# Autodesk Inventor assembly: enix_assembly_v2
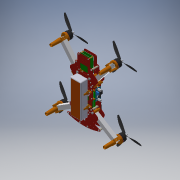
[picture p0: Inventor's stored thumbnail of the model, 180x180]
Saved by Autodesk Inventor 2016 (Build 200138000, 138)
## iProperties
Created: 2016-09-22
Part Number: enix_assembly_v2
Document SubType Name: Assembly
Designer: Jakub
Mass: 927.837 g
Surface Area: 3050.91 cm^2
Volume: 369.328 cm^3
Density: 2.51223 g/cm^3
Author: Jakub
## Documents named in this file (31)
- C:\Users\Jakub\Documents\DATA BANK\Projekty\Dron\Enix\V3\enix_assembly_v3.iam
- C:\Users\Jakub\Documents\DATA BANK\Projekty\Dron\Enix\V3\baseplate.ipt
- C:\Users\Jakub\Documents\DATA BANK\Projekty\Dron\Enix\V3\arm_grip.ipt
- C:\Users\Jakub\Documents\DATA BANK\Projekty\Dron\Enix\V3\arm_grip_mirror.ipt
- C:\Users\Jakub\Documents\DATA BANK\Projekty\Dron\Enix\V3\arm_lock.ipt
- C:\Users\Jakub\Documents\DATA BANK\Projekty\Dron\Enix\V3\dist25mm.ipt
- C:\Users\Jakub\Documents\Inventor\Content Center Files\R2016\en-US\AS 1427(04)\AS 1427 - M2 x 8(5) I.ipt
- C:\Users\Jakub\Documents\Inventor\Content Center Files\R2016\en-US\AS 1112 (2)\AS 1112 - M2  Type 5.ipt
- C:\Users\Jakub\Documents\DATA BANK\Projekty\Dron\Enix\V3\top_plate.ipt
- C:\Users\Jakub\Documents\Inventor\Content Center Files\R2016\en-US\UNI 6107\UNI 6107 - M4 x  30.ipt
- C:\Users\Jakub\Documents\Inventor\Content Center Files\R2016\en-US\ANSI B18.2.4.2M\ANSI B18.2.4.2M - M4x0,7 - 7.ipt
- C:\Users\Jakub\Documents\Inventor\Content Center Files\R2016\en-US\AS 1427(05)\AS 1427 - M3 x 5(5) II.ipt
- C:\Users\Jakub\Documents\DATA BANK\Projekty\Dron\Enix\V3\regulator.ipt
- C:\Users\Jakub\Documents\DATA BANK\Projekty\Dron\Enix\V3\dist10mmM2.ipt
- C:\Users\Jakub\Documents\DATA BANK\Projekty\Dron\Enix\V3\RASPBERRY PI 3.ipt
- C:\Users\Jakub\Documents\DATA BANK\Projekty\Dron\Enix\V3\dist5mmM2.ipt
- C:\Users\Jakub\Documents\DATA BANK\Projekty\Dron\Enix\V3\kamera.ipt
- C:\Users\Jakub\Documents\DATA BANK\Projekty\Dron\Enix\V3\cam_holder.ipt
- C:\Users\Jakub\Documents\DATA BANK\Projekty\Dron\Enix\V3\arm_front_rect.ipt
- C:\Users\Jakub\Documents\DATA BANK\Projekty\Dron\Enix\V3\arm_back_rect.ipt
- C:\Users\Jakub\Documents\DATA BANK\Projekty\Dron\Enix\V3\motor_mount.ipt
- C:\Users\Jakub\Documents\DATA BANK\Projekty\Dron\Enix\V3\motor_mount_lock.ipt
- C:\Users\Jakub\Documents\DATA BANK\Projekty\Dron\Enix\V3\Emax Rs2205 v1.ipt
- C:\Users\Jakub\Documents\DATA BANK\Projekty\Dron\Enix\V3\5x3_prop.ipt
- C:\Users\Jakub\Documents\DATA BANK\Projekty\Dron\Enix\V3\logic_conventer_lock.ipt
- C:\Users\Jakub\Documents\DATA BANK\Projekty\Dron\Enix\V3\altimuv3.iam
- C:\Users\Jakub\Documents\DATA BANK\Projekty\Dron\Enix\V3\kamamiLogicVoltageConverter\converter.iam
- C:\Users\Jakub\Documents\DATA BANK\Projekty\Dron\Enix\V3\kamamiTransformer\transformer.iam
- C:\Users\Jakub\Documents\DATA BANK\Projekty\Dron\Enix\V3\transformer_mount.ipt
- C:\Users\Jakub\Documents\DATA BANK\Projekty\Dron\Enix\V3\battery_distancer.ipt
- C:\Users\Jakub\Documents\DATA BANK\Projekty\Dron\Enix\V3\battery_vant_4500_4s.ipt
## Components (217 placed, 30 different names)
1. baseplate:1 — back_right_rot, front_right_rot, back_left_rot, front_left_rot, Mate:5, Mate:6, Mate:7, Mate:11, Mate:12, Mate:13, Mate:14, Mate:15, Mate:16, Mate:17, Mate:18, Mate:19, Mate:20, Mate:21, Mate:22, Mate:23, Mate:24, Mate:25, Mate:26, Mate:27, Mate:28, Mate:29, Mate:30, Mate:31, Mate:48, Mate:49, Mate:50, Mate:51, Mate:52, Mate:53, Mate:54, Mate:55, Mate:57, Mate:64, Mate:65, Mate:66, Mate:67, Mate:68, Mate:69, Mate:70, Mate:71, Mate:84, Mate:85, Mate:86, Mate:87, Mate:156, Mate:157, Mate:158, Mate:159, Mate:160, Mate:161, Mate:162, Mate:163, Mate:164, Mate:165, Mate:166, Mate:167, Mate:168, Mate:169, Mate:170, Mate:171, Mate:172, Mate:173, Mate:174, Mate:175, Mate:280, Mate:281, Mate:282, Mate:283, Mate:284, Mate:285, Mate:298, Mate:299, Mate:300, Mate:313, Mate:314, Mate:315, Mate:328, Mate:329, Mate:409, Mate:410, Mate:415, Mate:417, Mate:418, Mate:428, Mate:430, Mate:431, Mate:432, Mate:433, Mate:437, Mate:438, Mate:439, Mate:440, Mate:443, Mate:444, Mate:445, Mate:446, Mate:447, Mate:448, Mate:449, Mate:450, Mate:451, Mate:452, Mate:453, Mate:454, Mate:508, Mate:509, Mate:510, Mate:511, Mate:528, Mate:530, Mate:532, Mate:533, Mate:534, Mate:535, Mate:536, Mate:537, Mate:538, Mate:539, Mate:540, Mate:541, Mate:542, Mate:543, Mate:544, Mate:545
2. arm_grip:1 — back_right_rot, Mate:76, Mate:344, Mate:346, Angle:1
3. arm_grip:2 — front_right_rot, Mate:77, Mate:340, Mate:349, Angle:4
4. arm_grip_mirror:1 — back_left_rot, Mate:79, Mate:345, Mate:347, Angle:2
5. arm_grip_mirror:2 — front_left_rot, Mate:78, Mate:341, Mate:348, Angle:3
6. arm_lock:1 — Mate:5, Mate:6, Mate:7, Mate:32, Mate:33, Mate:38, Mate:39
7. arm_lock:2 — Mate:11, Mate:12, Mate:13, Mate:40, Mate:41, Mate:46, Mate:47
8. arm_lock:3 — Mate:14, Mate:15, Mate:16, Mate:42, Mate:43, Mate:44, Mate:45
9. arm_lock:4 — Mate:17, Mate:18, Mate:19, Mate:34, Mate:35, Mate:36, Mate:37
10. dist25mm:1 — Mate:20, Mate:23
11. dist25mm:2 — Mate:21, Mate:22
12. dist25mm:3 — Mate:27, Mate:28
13. dist25mm:4 — Mate:26, Mate:29
14. dist25mm:5 — Mate:25, Mate:30
15. dist25mm:6 — Mate:24, Mate:31, Mate:72, Mate:73
16. AS 1427 H - Metric M2 x 8:1 — Mate:32, Mate:38
17. AS 1427 H - Metric M2 x 8:2 — Mate:33, Mate:39, Mate:56
18. AS 1427 H - Metric M2 x 8:3 — Mate:34, Mate:36, Mate:63
19. AS 1427 H - Metric M2 x 8:4 — Mate:35, Mate:37, Mate:62
20. AS 1427 H - Metric M2 x 8:5 — Mate:42, Mate:44, Mate:60
21. AS 1427 H - Metric M2 x 8:6 — Mate:43, Mate:45, Mate:61
22. AS 1427 H - Metric M2 x 8:7 — Mate:41, Mate:46, Mate:58
23. AS 1427 H - Metric M2 x 8:8 — Mate:40, Mate:47, Mate:59
24. AS 1112 (2) - Metric M2  Type 5:1 — Mate:55, Mate:62
25. AS 1112 (2) - Metric M2  Type 5:2 — Mate:54, Mate:61
26. AS 1112 (2) - Metric M2  Type 5:3 — Mate:53, Mate:60
27. AS 1112 (2) - Metric M2  Type 5:4 — Mate:52, Mate:56
28. AS 1112 (2) - Metric M2  Type 5:5 — Mate:51, Mate:58
29. AS 1112 (2) - Metric M2  Type 5:6 — Mate:50, Mate:57
30. AS 1112 (2) - Metric M2  Type 5:7 — Mate:49, Mate:59
31. AS 1112 (2) - Metric M2  Type 5:8 — Mate:48, Mate:63
32. dist25mm:7 — Mate:68, Mate:69
33. dist25mm:8 — Mate:70, Mate:71, Mate:74
34. dist25mm:9 — Mate:66, Mate:67, Mate:75
35. dist25mm:10 — Mate:64, Mate:65
36. top_plate:1 — Mate:72, Mate:73, Mate:74, Mate:75, Mate:80, Mate:81, Mate:82, Mate:83, Mate:92, Mate:93, Mate:94, Mate:95, Mate:96, Mate:97, Mate:98, Mate:99, Mate:100, Mate:101, Mate:102, Mate:103, Mate:104, Mate:105, Mate:106, Mate:107, Mate:108, Mate:109, Mate:110, Mate:111, Mate:112, Mate:113, Mate:114, Mate:115, Mate:116, Mate:117, Mate:118, Mate:119, Mate:136, Mate:137, Mate:138, Mate:139, Mate:140, Mate:141, Mate:142, Mate:143, Mate:144, Mate:145, Mate:146, Mate:147, Mate:148, Mate:149, Mate:150, Mate:151, Mate:152, Mate:153, Mate:154, Mate:155, Mate:219, Mate:220, Mate:221, Mate:222, Mate:223, Mate:224, Mate:225, Mate:226, Mate:249, Mate:250, Mate:251, Mate:252, Mate:419, Mate:420, Mate:421, Mate:422, Mate:425, Mate:426, Mate:484, Mate:485, Mate:492, Mate:493, Mate:496, Mate:497, Mate:502, Mate:503, Mate:504, Mate:505
37. UNI 6107 M4 x  30:1 — Mate:76, Mate:81, Mate:89
38. UNI 6107 M4 x  30:2 — Mate:77, Mate:82, Mate:90
39. UNI 6107 M4 x  30:3 — Mate:78, Mate:83, Mate:91
40. UNI 6107 M4 x  30:4 — Mate:79, Mate:80, Mate:88
41. ANSI B18.2.4.2M M4x0,7:5 — Mate:87, Mate:91
42. ANSI B18.2.4.2M M4x0,7:6 — Mate:86, Mate:90
43. ANSI B18.2.4.2M M4x0,7:7 — Mate:85, Mate:88
44. ANSI B18.2.4.2M M4x0,7:8 — Mate:84, Mate:89
45. arm_lock:5 — Mate:92, Mate:93, Mate:94, Mate:132, Mate:133
46. arm_lock:6 — Mate:95, Mate:96, Mate:97, Mate:128, Mate:129
47. arm_lock:7 — Mate:98, Mate:99, Mate:100, Mate:120, Mate:121
48. arm_lock:8 — Mate:101, Mate:102, Mate:103, Mate:124, Mate:125
49. AS 1427 H - Metric M2 x 8:9 — Mate:108, Mate:118, Mate:131
50. AS 1427 H - Metric M2 x 8:10 — Mate:107, Mate:113, Mate:127
51. AS 1427 H - Metric M2 x 8:11 — Mate:109, Mate:119, Mate:130
52. AS 1427 H - Metric M2 x 8:12 — Mate:106, Mate:112, Mate:126
53. AS 1427 H - Metric M2 x 8:13 — Mate:110, Mate:117, Mate:135
54. AS 1427 H - Metric M2 x 8:14 — Mate:105, Mate:114, Mate:123
55. AS 1427 H - Metric M2 x 8:15 — Mate:111, Mate:116, Mate:134
56. AS 1427 H - Metric M2 x 8:16 — Mate:104, Mate:115, Mate:122
57. AS 1112 (2) - Metric M2  Type 5:9 — Mate:120, Mate:123
58. AS 1112 (2) - Metric M2  Type 5:10 — Mate:121, Mate:122
59. AS 1112 (2) - Metric M2  Type 5:11 — Mate:124, Mate:127
60. AS 1112 (2) - Metric M2  Type 5:12 — Mate:125, Mate:126
61. AS 1112 (2) - Metric M2  Type 5:13 — Mate:133, Mate:134
62. AS 1112 (2) - Metric M2  Type 5:14 — Mate:132, Mate:135
63. AS 1112 (2) - Metric M2  Type 5:15 — Mate:129, Mate:131
64. AS 1112 (2) - Metric M2  Type 5:16 — Mate:128, Mate:130
65. AS 1427 H - Metric M3 x 5:1 — Mate:137, Mate:145
66. AS 1427 H - Metric M3 x 5:2 — Mate:138, Mate:146
67. AS 1427 H - Metric M3 x 5:3 — Mate:154, Mate:155
68. AS 1427 H - Metric M3 x 5:4 — Mate:144, Mate:153
69. AS 1427 H - Metric M3 x 5:5 — Mate:143, Mate:151
70. AS 1427 H - Metric M3 x 5:6 — Mate:142, Mate:152
71. AS 1427 H - Metric M3 x 5:7 — Mate:141, Mate:149
72. AS 1427 H - Metric M3 x 5:8 — Mate:140, Mate:148
73. AS 1427 H - Metric M3 x 5:9 — Mate:139, Mate:147
74. AS 1427 H - Metric M3 x 5:10 — Mate:136, Mate:150
75. AS 1427 H - Metric M3 x 5:11 — Mate:165, Mate:166
76. AS 1427 H - Metric M3 x 5:12 — Mate:164, Mate:167
77. AS 1427 H - Metric M3 x 5:13 — Mate:163, Mate:168
78. AS 1427 H - Metric M3 x 5:14 — Mate:162, Mate:169
79. AS 1427 H - Metric M3 x 5:15 — Mate:161, Mate:170
80. AS 1427 H - Metric M3 x 5:16 — Mate:160, Mate:171
81. AS 1427 H - Metric M3 x 5:17 — Mate:159, Mate:172
82. AS 1427 H - Metric M3 x 5:18 — Mate:158, Mate:173
83. AS 1427 H - Metric M3 x 5:19 — Mate:157, Mate:175
84. AS 1427 H - Metric M3 x 5:20 — Mate:156, Mate:174
85. RASPBERRY PI 3:1 — Mate:227, Mate:228, Mate:229, Mate:230, Mate:243, Mate:244, Mate:245, Mate:246
86. dist5mmM2:2 — Mate:221, Mate:225, Mate:228, Mate:240, Mate:253
87. dist5mmM2:3 — Mate:220, Mate:226, Mate:227, Mate:229, Mate:241, Mate:256
88. dist5mmM2:4 — Mate:219, Mate:223, Mate:230, Mate:242, Mate:255
89. dist5mmM2:5 — Mate:222, Mate:224, Mate:239, Mate:254
90. AS 1427 H - Metric M2 x 8:17 — Mate:239, Mate:243
91. AS 1427 H - Metric M2 x 8:18 — Mate:240, Mate:244
92. AS 1427 H - Metric M2 x 8:19 — Mate:241, Mate:245
93. AS 1427 H - Metric M2 x 8:20 — Mate:242, Mate:246
94. AS 1112 (2) - Metric M2  Type 5:20 — Mate:249, Mate:253
95. AS 1112 (2) - Metric M2  Type 5:21 — Mate:250, Mate:254
96. AS 1112 (2) - Metric M2  Type 5:22 — Mate:251, Mate:256
97. AS 1112 (2) - Metric M2  Type 5:23 — Mate:252, Mate:255
98. dist5mmM2:6 — Mate:282, Mate:284, Mate:302, Mate:459
99. dist5mmM2:7 — Mate:281, Mate:283, Mate:301
100. dist5mmM2:8 — Mate:280, Mate:285, Mate:303
101. dist10mmM2:7
102. dist10mmM2:8
103. dist10mmM2:9 — Mate:461
104. AS 1112 (2) - Metric M2  Type 5:24 — Mate:298, Mate:302
105. AS 1112 (2) - Metric M2  Type 5:25 — Mate:300, Mate:303
106. AS 1112 (2) - Metric M2  Type 5:26 — Mate:299, Mate:301
107. AS 1427 H - Metric M2 x 8:21 — Mate:462
108. AS 1427 H - Metric M2 x 8:22
109. AS 1427 H - Metric M2 x 8:23
110. kamera:1 — Mate:310, Mate:311, Mate:312, Mate:320, Mate:321, Mate:322, Mate:323, Mate:324, Mate:325, Mate:326, Mate:327
111. cam_holder:1 — Mate:310, Mate:311, Mate:312, Mate:313, Mate:314, Mate:315, Mate:316, Mate:317, Mate:318, Mate:319, Mate:332, Mate:333, Mate:334, Mate:335
112. AS 1427 H - Metric M2 x 8:24 — Mate:317, Mate:319, Mate:330
113. AS 1427 H - Metric M2 x 8:25 — Mate:326, Mate:327, Mate:339
114. AS 1427 H - Metric M2 x 8:26 — Mate:324, Mate:325, Mate:338
115. AS 1427 H - Metric M2 x 8:27 — Mate:320, Mate:321, Mate:336
116. AS 1427 H - Metric M2 x 8:28 — Mate:316, Mate:318, Mate:331
117. AS 1427 H - Metric M2 x 8:29 — Mate:322, Mate:323, Mate:337
118. AS 1112 (2) - Metric M2  Type 5:27 — Mate:329, Mate:330
119. AS 1112 (2) - Metric M2  Type 5:28 — Mate:328, Mate:331
120. AS 1112 (2) - Metric M2  Type 5:29 — Mate:332, Mate:339
121. AS 1112 (2) - Metric M2  Type 5:30 — Mate:333, Mate:338
122. AS 1112 (2) - Metric M2  Type 5:31 — Mate:334, Mate:337
123. AS 1112 (2) - Metric M2  Type 5:32 — Mate:335, Mate:336
124. arm_front_rect:1 — Mate:340, Mate:349, Angle:4, Mate:350, Mate:356, Angle:8, Mate:361, Mate:371
125. arm_front_rect:2 — Mate:341, Mate:348, Angle:3, Mate:351, Mate:357, Angle:7, Mate:358, Mate:377
126. arm_back_rect:1 — Mate:344, Mate:346, Angle:1, Mate:352, Mate:355, Angle:6, Mate:364, Mate:376
127. arm_back_rect:2 — Mate:345, Mate:347, Angle:2, Mate:353, Mate:354, Angle:5, Mate:367, Mate:375
128. motor_mount:1 — Mate:350, Mate:356, Angle:8, Mate:362, Mate:363, Mate:370
129. motor_mount:2 — Mate:351, Mate:357, Angle:7, Mate:359, Mate:360, Mate:372
130. motor_mount:3 — Mate:353, Mate:354, Angle:5, Mate:368, Mate:369, Mate:374
131. motor_mount:4 — Mate:352, Mate:355, Angle:6, Mate:365, Mate:366, Mate:373
132. motor_mount_lock:1 — Mate:358, Mate:359, Mate:360
133. motor_mount_lock:2 — Mate:361, Mate:362, Mate:363
134. motor_mount_lock:3 — Mate:364, Mate:365, Mate:366
135. motor_mount_lock:4 — Mate:367, Mate:368, Mate:369
136. Emax Rs2205 v1:1 — Mate:372, Mate:377, Mate:379, Mate:384
137. Emax Rs2205 v1:2 — Mate:370, Mate:371, Mate:378, Mate:382
138. Emax Rs2205 v1:3 — Mate:373, Mate:376, Mate:381, Mate:383
139. Emax Rs2205 v1:4 — Mate:374, Mate:375, Mate:380, Mate:385
140. 5x3_prop:1 — Mate:380, Mate:385
141. 5x3_prop:2 — Mate:379, Mate:384
142. 5x3_prop:3 — Mate:378, Mate:382
143. 5x3_prop:4 — Mate:381, Mate:383
144. dist5mmM2:9 — Mate:409, Mate:410, Mate:412, Mate:414, Mate:416
145. dist10mmM2:12 — Mate:412, Mate:460
146. AS 1427 H - Metric M2 x 8:30 — Mate:414
147. AS 1112 (2) - Metric M2  Type 5:34 — Mate:415, Mate:416
148. logic_conventer_lock:1 — Mate:417, Mate:418, Flush:1, Mate:429, Mate:524, Mate:525, Mate:526, Mate:527
149. altimuv3:1 [sub-assembly] — Mate:427, Mate:486, Mate:487, Mate:488, Mate:489, Mate:490, Mate:491
150. dist5mmM2:10 — Mate:419, Mate:421, Mate:424, Mate:484
151. dist5mmM2:11 — Mate:420, Mate:422, Mate:423, Mate:427, Mate:485, Mate:486, Mate:487
152. AS 1112 (2) - Metric M2  Type 5:35 — Mate:423, Mate:425
153. AS 1112 (2) - Metric M2  Type 5:36 — Mate:424, Mate:426
154. converter:1 [sub-assembly] — Mate:428, Flush:1, Mate:429
155. transformer_mount:1 — Mate:430, Mate:431, Mate:434, Mate:435, Mate:499, Mate:500, Mate:518
156. transformer_mount:2 — Mate:432, Mate:433, Mate:436, Mate:498, Mate:501, Mate:516
157. transformer:1 [sub-assembly] — Mate:434, Mate:435, Mate:436, Mate:556, Mate:557, Mate:558, Mate:559
158. transformer_mount:3 — Mate:437, Mate:439, Mate:441, Mate:442, Mate:494, Mate:506, Mate:520
159. transformer_mount:4 — Mate:438, Mate:440, Mate:495, Mate:507, Mate:522
160. transformer:2 [sub-assembly] — Mate:441, Mate:442, Mate:560, Mate:561, Mate:562, Mate:563
161. dist5mmM2:12 — Mate:445, Mate:450, Mate:458
162. dist5mmM2:13 — Mate:443, Mate:447, Mate:456, Mate:464
163. dist5mmM2:14 — Mate:446, Mate:449, Mate:455
164. dist5mmM2:15 — Mate:444, Mate:448, Mate:457, Mate:463
165. AS 1112 (2) - Metric M2  Type 5:37 — Mate:454, Mate:455
166. AS 1112 (2) - Metric M2  Type 5:38 — Mate:453, Mate:457
167. AS 1112 (2) - Metric M2  Type 5:39 — Mate:452, Mate:458
168. AS 1112 (2) - Metric M2  Type 5:40 — Mate:451, Mate:456
169. regulator:1 — Mate:459, Mate:460
170. regulator:2 — Mate:461, Mate:462
171. regulator:3 — Mate:463, Mate:464, Mate:465, Mate:466, Mate:467, Mate:468, Mate:469, Mate:470, Mate:471, Mate:472
172. regulator:4 — Mate:473, Mate:474, Mate:475, Mate:476, Mate:477, Mate:478, Mate:479, Mate:480, Mate:481, Mate:482, Mate:483
173. dist10mmM2:13 — Mate:467, Mate:472
174. dist10mmM2:14 — Mate:466, Mate:470, Mate:474
175. dist10mmM2:15 — Mate:465, Mate:469, Mate:473, Mate:475
176. dist10mmM2:16 — Mate:468, Mate:471
177. AS 1427 H - Metric M2 x 8:31 — Mate:479, Mate:483
178. AS 1427 H - Metric M2 x 8:32 — Mate:476, Mate:481
179. AS 1427 H - Metric M2 x 8:33 — Mate:477, Mate:480
180. AS 1427 H - Metric M2 x 8:34 — Mate:478, Mate:482
181. AS 1427 H - Metric M2 x 8:35 — Mate:488, Mate:491
182. AS 1427 H - Metric M2 x 8:36 — Mate:489, Mate:490
183. AS 1427 H - Metric M2 x 8:37 — Mate:495, Mate:507, Mate:514
184. AS 1427 H - Metric M2 x 8:38 — Mate:493, Mate:505, Mate:523
185. AS 1427 H - Metric M2 x 8:39 — Mate:492, Mate:504, Mate:521
186. AS 1427 H - Metric M2 x 8:40 — Mate:494, Mate:506, Mate:515
187. AS 1427 H - Metric M2 x 8:41 — Mate:499, Mate:500, Mate:512
188. AS 1427 H - Metric M2 x 8:42 — Mate:498, Mate:501, Mate:513
189. AS 1427 H - Metric M2 x 8:43 — Mate:496, Mate:503, Mate:519
190. AS 1427 H - Metric M2 x 8:44 — Mate:497, Mate:502, Mate:517
191. AS 1112 (2) - Metric M2  Type 5:41 — Mate:508, Mate:514
192. AS 1112 (2) - Metric M2  Type 5:42 — Mate:510, Mate:515
193. AS 1112 (2) - Metric M2  Type 5:43 — Mate:511, Mate:512
194. AS 1112 (2) - Metric M2  Type 5:44 — Mate:509, Mate:513
195. AS 1112 (2) - Metric M2  Type 5:45 — Mate:522, Mate:523
196. AS 1112 (2) - Metric M2  Type 5:46 — Mate:520, Mate:521
197. AS 1112 (2) - Metric M2  Type 5:47 — Mate:518, Mate:519
198. AS 1112 (2) - Metric M2  Type 5:48 — Mate:516, Mate:517
199. AS 1427 H - Metric M2 x 8:45 — Mate:524, Mate:527, Mate:531
200. AS 1427 H - Metric M2 x 8:46 — Mate:525, Mate:526, Mate:529
201. AS 1112 (2) - Metric M2  Type 5:49 — Mate:530, Mate:531
202. AS 1112 (2) - Metric M2  Type 5:50 — Mate:528, Mate:529
203. battery_distancer:1 — Mate:532, Mate:533, Mate:534, Mate:548, Mate:550
204. battery_distancer:2 — Mate:535, Mate:536, Mate:537, Mate:546, Mate:552, Mate:554, Mate:555
205. AS 1427 H - Metric M2 x 8:47 — Mate:538, Mate:539, Mate:553
206. AS 1427 H - Metric M2 x 8:48 — Mate:540, Mate:541, Mate:551
207. AS 1427 H - Metric M2 x 8:49 — Mate:543, Mate:544, Mate:549
208. AS 1427 H - Metric M2 x 8:50 — Mate:542, Mate:545, Mate:547
209. AS 1112 (2) - Metric M2  Type 5:51 — Mate:552, Mate:553
210. AS 1112 (2) - Metric M2  Type 5:52 — Mate:550, Mate:551
211. AS 1112 (2) - Metric M2  Type 5:53 — Mate:548, Mate:549
212. AS 1112 (2) - Metric M2  Type 5:54 — Mate:546, Mate:547
213. battery_vant_4500_4s:1 — Mate:554, Mate:555
214. AS 1427 H - Metric M2 x 8:51 — Mate:556, Mate:559
215. AS 1427 H - Metric M2 x 8:52 — Mate:557, Mate:558
216. AS 1427 H - Metric M2 x 8:53 — Mate:561, Mate:562
217. AS 1427 H - Metric M2 x 8:54 — Mate:560, Mate:563
## Relationships (448: Mate 435, Angle 8, RevoluteJoint 4, Flush 1)
- back_right_rot [RevoluteJoint]: baseplate:1 ↔ arm_grip:1
- front_right_rot [RevoluteJoint]: baseplate:1 ↔ arm_grip:2
- back_left_rot [RevoluteJoint]: baseplate:1 ↔ arm_grip_mirror:1
- front_left_rot [RevoluteJoint]: baseplate:1 ↔ arm_grip_mirror:2
- Mate:5: baseplate:1 ↔ arm_lock:1
- Mate:6: baseplate:1 ↔ arm_lock:1
- Mate:7: baseplate:1 ↔ arm_lock:1
- Mate:11: baseplate:1 ↔ arm_lock:2
- Mate:12: baseplate:1 ↔ arm_lock:2
- Mate:13: baseplate:1 ↔ arm_lock:2
- Mate:14: baseplate:1 ↔ arm_lock:3
- Mate:15: baseplate:1 ↔ arm_lock:3
- Mate:16: baseplate:1 ↔ arm_lock:3
- Mate:17: baseplate:1 ↔ arm_lock:4
- Mate:18: baseplate:1 ↔ arm_lock:4
- Mate:19: baseplate:1 ↔ arm_lock:4
- Mate:20: baseplate:1 ↔ dist25mm:1
- Mate:21: baseplate:1 ↔ dist25mm:2
- Mate:22: baseplate:1 ↔ dist25mm:2
- Mate:23: baseplate:1 ↔ dist25mm:1
- Mate:24: baseplate:1 ↔ dist25mm:6
- Mate:25: baseplate:1 ↔ dist25mm:5
- Mate:26: baseplate:1 ↔ dist25mm:4
- Mate:27: baseplate:1 ↔ dist25mm:3
- Mate:28: baseplate:1 ↔ dist25mm:3
- Mate:29: baseplate:1 ↔ dist25mm:4
- Mate:30: baseplate:1 ↔ dist25mm:5
- Mate:31: baseplate:1 ↔ dist25mm:6
- Mate:32: arm_lock:1 ↔ AS 1427 H - Metric M2 x 8:1
- Mate:33: arm_lock:1 ↔ AS 1427 H - Metric M2 x 8:2
- Mate:34: arm_lock:4 ↔ AS 1427 H - Metric M2 x 8:3
- Mate:35: arm_lock:4 ↔ AS 1427 H - Metric M2 x 8:4
- Mate:36: arm_lock:4 ↔ AS 1427 H - Metric M2 x 8:3
- Mate:37: arm_lock:4 ↔ AS 1427 H - Metric M2 x 8:4
- Mate:38: arm_lock:1 ↔ AS 1427 H - Metric M2 x 8:1
- Mate:39: arm_lock:1 ↔ AS 1427 H - Metric M2 x 8:2
- Mate:40: arm_lock:2 ↔ AS 1427 H - Metric M2 x 8:8
- Mate:41: arm_lock:2 ↔ AS 1427 H - Metric M2 x 8:7
- Mate:42: arm_lock:3 ↔ AS 1427 H - Metric M2 x 8:5
- Mate:43: arm_lock:3 ↔ AS 1427 H - Metric M2 x 8:6
- Mate:44: arm_lock:3 ↔ AS 1427 H - Metric M2 x 8:5
- Mate:45: arm_lock:3 ↔ AS 1427 H - Metric M2 x 8:6
- Mate:46: arm_lock:2 ↔ AS 1427 H - Metric M2 x 8:7
- Mate:47: arm_lock:2 ↔ AS 1427 H - Metric M2 x 8:8
- Mate:48: baseplate:1 ↔ AS 1112 (2) - Metric M2  Type 5:8
- Mate:49: baseplate:1 ↔ AS 1112 (2) - Metric M2  Type 5:7
- Mate:50: baseplate:1 ↔ AS 1112 (2) - Metric M2  Type 5:6
- Mate:51: baseplate:1 ↔ AS 1112 (2) - Metric M2  Type 5:5
- Mate:52: baseplate:1 ↔ AS 1112 (2) - Metric M2  Type 5:4
- Mate:53: baseplate:1 ↔ AS 1112 (2) - Metric M2  Type 5:3
- Mate:54: baseplate:1 ↔ AS 1112 (2) - Metric M2  Type 5:2
- Mate:55: baseplate:1 ↔ AS 1112 (2) - Metric M2  Type 5:1
- Mate:56: AS 1427 H - Metric M2 x 8:2 ↔ AS 1112 (2) - Metric M2  Type 5:4
- Mate:57: baseplate:1 ↔ AS 1112 (2) - Metric M2  Type 5:6
- Mate:58: AS 1427 H - Metric M2 x 8:7 ↔ AS 1112 (2) - Metric M2  Type 5:5
- Mate:59: AS 1427 H - Metric M2 x 8:8 ↔ AS 1112 (2) - Metric M2  Type 5:7
- Mate:60: AS 1427 H - Metric M2 x 8:5 ↔ AS 1112 (2) - Metric M2  Type 5:3
- Mate:61: AS 1427 H - Metric M2 x 8:6 ↔ AS 1112 (2) - Metric M2  Type 5:2
- Mate:62: AS 1427 H - Metric M2 x 8:4 ↔ AS 1112 (2) - Metric M2  Type 5:1
- Mate:63: AS 1427 H - Metric M2 x 8:3 ↔ AS 1112 (2) - Metric M2  Type 5:8
- Mate:64: baseplate:1 ↔ dist25mm:10
- Mate:65: baseplate:1 ↔ dist25mm:10
- Mate:66: baseplate:1 ↔ dist25mm:9
- Mate:67: baseplate:1 ↔ dist25mm:9
- Mate:68: baseplate:1 ↔ dist25mm:7
- Mate:69: baseplate:1 ↔ dist25mm:7
- Mate:70: baseplate:1 ↔ dist25mm:8
- Mate:71: baseplate:1 ↔ dist25mm:8
- Mate:72: dist25mm:6 ↔ top_plate:1
- Mate:73: dist25mm:6 ↔ top_plate:1
- Mate:74: dist25mm:8 ↔ top_plate:1
- Mate:75: dist25mm:9 ↔ top_plate:1
- Mate:76: arm_grip:1 ↔ UNI 6107 M4 x  30:1
- Mate:77: arm_grip:2 ↔ UNI 6107 M4 x  30:2
- Mate:78: arm_grip_mirror:2 ↔ UNI 6107 M4 x  30:3
- Mate:79: arm_grip_mirror:1 ↔ UNI 6107 M4 x  30:4
- Mate:80: top_plate:1 ↔ UNI 6107 M4 x  30:4
- Mate:81: top_plate:1 ↔ UNI 6107 M4 x  30:1
- Mate:82: top_plate:1 ↔ UNI 6107 M4 x  30:2
- Mate:83: top_plate:1 ↔ UNI 6107 M4 x  30:3
- Mate:84: baseplate:1 ↔ ANSI B18.2.4.2M M4x0,7:8
- Mate:85: baseplate:1 ↔ ANSI B18.2.4.2M M4x0,7:7
- Mate:86: baseplate:1 ↔ ANSI B18.2.4.2M M4x0,7:6
- Mate:87: baseplate:1 ↔ ANSI B18.2.4.2M M4x0,7:5
- Mate:88: UNI 6107 M4 x  30:4 ↔ ANSI B18.2.4.2M M4x0,7:7
- Mate:89: UNI 6107 M4 x  30:1 ↔ ANSI B18.2.4.2M M4x0,7:8
- Mate:90: UNI 6107 M4 x  30:2 ↔ ANSI B18.2.4.2M M4x0,7:6
- Mate:91: UNI 6107 M4 x  30:3 ↔ ANSI B18.2.4.2M M4x0,7:5
- Mate:92: top_plate:1 ↔ arm_lock:5
- Mate:93: top_plate:1 ↔ arm_lock:5
- Mate:94: top_plate:1 ↔ arm_lock:5
- Mate:95: top_plate:1 ↔ arm_lock:6
- Mate:96: top_plate:1 ↔ arm_lock:6
- Mate:97: top_plate:1 ↔ arm_lock:6
- Mate:98: top_plate:1 ↔ arm_lock:7
- Mate:99: top_plate:1 ↔ arm_lock:7
- Mate:100: top_plate:1 ↔ arm_lock:7
- Mate:101: top_plate:1 ↔ arm_lock:8
- Mate:102: top_plate:1 ↔ arm_lock:8
- Mate:103: top_plate:1 ↔ arm_lock:8
- Mate:104: top_plate:1 ↔ AS 1427 H - Metric M2 x 8:16
- Mate:105: top_plate:1 ↔ AS 1427 H - Metric M2 x 8:14
- Mate:106: top_plate:1 ↔ AS 1427 H - Metric M2 x 8:12
- Mate:107: top_plate:1 ↔ AS 1427 H - Metric M2 x 8:10
- Mate:108: top_plate:1 ↔ AS 1427 H - Metric M2 x 8:9
- Mate:109: top_plate:1 ↔ AS 1427 H - Metric M2 x 8:11
- Mate:110: top_plate:1 ↔ AS 1427 H - Metric M2 x 8:13
- Mate:111: top_plate:1 ↔ AS 1427 H - Metric M2 x 8:15
- Mate:112: top_plate:1 ↔ AS 1427 H - Metric M2 x 8:12
- Mate:113: top_plate:1 ↔ AS 1427 H - Metric M2 x 8:10
- Mate:114: top_plate:1 ↔ AS 1427 H - Metric M2 x 8:14
- Mate:115: top_plate:1 ↔ AS 1427 H - Metric M2 x 8:16
- Mate:116: top_plate:1 ↔ AS 1427 H - Metric M2 x 8:15
- Mate:117: top_plate:1 ↔ AS 1427 H - Metric M2 x 8:13
- Mate:118: top_plate:1 ↔ AS 1427 H - Metric M2 x 8:9
- Mate:119: top_plate:1 ↔ AS 1427 H - Metric M2 x 8:11
- Mate:120: arm_lock:7 ↔ AS 1112 (2) - Metric M2  Type 5:9
- Mate:121: arm_lock:7 ↔ AS 1112 (2) - Metric M2  Type 5:10
- Mate:122: AS 1427 H - Metric M2 x 8:16 ↔ AS 1112 (2) - Metric M2  Type 5:10
- Mate:123: AS 1427 H - Metric M2 x 8:14 ↔ AS 1112 (2) - Metric M2  Type 5:9
- Mate:124: arm_lock:8 ↔ AS 1112 (2) - Metric M2  Type 5:11
- Mate:125: arm_lock:8 ↔ AS 1112 (2) - Metric M2  Type 5:12
- Mate:126: AS 1427 H - Metric M2 x 8:12 ↔ AS 1112 (2) - Metric M2  Type 5:12
- Mate:127: AS 1427 H - Metric M2 x 8:10 ↔ AS 1112 (2) - Metric M2  Type 5:11
- Mate:128: arm_lock:6 ↔ AS 1112 (2) - Metric M2  Type 5:16
- Mate:129: arm_lock:6 ↔ AS 1112 (2) - Metric M2  Type 5:15
- Mate:130: AS 1427 H - Metric M2 x 8:11 ↔ AS 1112 (2) - Metric M2  Type 5:16
- Mate:131: AS 1427 H - Metric M2 x 8:9 ↔ AS 1112 (2) - Metric M2  Type 5:15
- Mate:132: arm_lock:5 ↔ AS 1112 (2) - Metric M2  Type 5:14
- Mate:133: arm_lock:5 ↔ AS 1112 (2) - Metric M2  Type 5:13
- Mate:134: AS 1427 H - Metric M2 x 8:15 ↔ AS 1112 (2) - Metric M2  Type 5:13
- Mate:135: AS 1427 H - Metric M2 x 8:13 ↔ AS 1112 (2) - Metric M2  Type 5:14
- Mate:136: top_plate:1 ↔ AS 1427 H - Metric M3 x 5:10
- Mate:137: top_plate:1 ↔ AS 1427 H - Metric M3 x 5:1
- Mate:138: top_plate:1 ↔ AS 1427 H - Metric M3 x 5:2
- Mate:139: top_plate:1 ↔ AS 1427 H - Metric M3 x 5:9
- Mate:140: top_plate:1 ↔ AS 1427 H - Metric M3 x 5:8
- Mate:141: top_plate:1 ↔ AS 1427 H - Metric M3 x 5:7
- Mate:142: top_plate:1 ↔ AS 1427 H - Metric M3 x 5:6
- Mate:143: top_plate:1 ↔ AS 1427 H - Metric M3 x 5:5
- Mate:144: top_plate:1 ↔ AS 1427 H - Metric M3 x 5:4
- Mate:145: top_plate:1 ↔ AS 1427 H - Metric M3 x 5:1
- Mate:146: top_plate:1 ↔ AS 1427 H - Metric M3 x 5:2
- Mate:147: top_plate:1 ↔ AS 1427 H - Metric M3 x 5:9
- Mate:148: top_plate:1 ↔ AS 1427 H - Metric M3 x 5:8
- Mate:149: top_plate:1 ↔ AS 1427 H - Metric M3 x 5:7
- Mate:150: top_plate:1 ↔ AS 1427 H - Metric M3 x 5:10
- Mate:151: top_plate:1 ↔ AS 1427 H - Metric M3 x 5:5
- Mate:152: top_plate:1 ↔ AS 1427 H - Metric M3 x 5:6
- Mate:153: top_plate:1 ↔ AS 1427 H - Metric M3 x 5:4
- Mate:154: top_plate:1 ↔ AS 1427 H - Metric M3 x 5:3
- Mate:155: top_plate:1 ↔ AS 1427 H - Metric M3 x 5:3
- Mate:156: baseplate:1 ↔ AS 1427 H - Metric M3 x 5:20
- Mate:157: baseplate:1 ↔ AS 1427 H - Metric M3 x 5:19
- Mate:158: baseplate:1 ↔ AS 1427 H - Metric M3 x 5:18
- Mate:159: baseplate:1 ↔ AS 1427 H - Metric M3 x 5:17
- Mate:160: baseplate:1 ↔ AS 1427 H - Metric M3 x 5:16
- Mate:161: baseplate:1 ↔ AS 1427 H - Metric M3 x 5:15
- Mate:162: baseplate:1 ↔ AS 1427 H - Metric M3 x 5:14
- Mate:163: baseplate:1 ↔ AS 1427 H - Metric M3 x 5:13
- Mate:164: baseplate:1 ↔ AS 1427 H - Metric M3 x 5:12
- Mate:165: baseplate:1 ↔ AS 1427 H - Metric M3 x 5:11
- Mate:166: baseplate:1 ↔ AS 1427 H - Metric M3 x 5:11
- Mate:167: baseplate:1 ↔ AS 1427 H - Metric M3 x 5:12
- Mate:168: baseplate:1 ↔ AS 1427 H - Metric M3 x 5:13
- Mate:169: baseplate:1 ↔ AS 1427 H - Metric M3 x 5:14
- Mate:170: baseplate:1 ↔ AS 1427 H - Metric M3 x 5:15
- Mate:171: baseplate:1 ↔ AS 1427 H - Metric M3 x 5:16
- Mate:172: baseplate:1 ↔ AS 1427 H - Metric M3 x 5:17
- Mate:173: baseplate:1 ↔ AS 1427 H - Metric M3 x 5:18
- Mate:174: baseplate:1 ↔ AS 1427 H - Metric M3 x 5:20
- Mate:175: baseplate:1 ↔ AS 1427 H - Metric M3 x 5:19
- Mate:219: top_plate:1 ↔ dist5mmM2:4
- Mate:220: top_plate:1 ↔ dist5mmM2:3
- Mate:221: top_plate:1 ↔ dist5mmM2:2
- Mate:222: top_plate:1 ↔ dist5mmM2:5
- Mate:223: top_plate:1 ↔ dist5mmM2:4
- Mate:224: top_plate:1 ↔ dist5mmM2:5
- Mate:225: top_plate:1 ↔ dist5mmM2:2
- Mate:226: top_plate:1 ↔ dist5mmM2:3
- Mate:227: RASPBERRY PI 3:1 ↔ dist5mmM2:3
- Mate:228: RASPBERRY PI 3:1 ↔ dist5mmM2:2
- Mate:229: RASPBERRY PI 3:1 ↔ dist5mmM2:3
- Mate:230: RASPBERRY PI 3:1 ↔ dist5mmM2:4
- Mate:239: dist5mmM2:5 ↔ AS 1427 H - Metric M2 x 8:17
- Mate:240: dist5mmM2:2 ↔ AS 1427 H - Metric M2 x 8:18
- Mate:241: dist5mmM2:3 ↔ AS 1427 H - Metric M2 x 8:19
- Mate:242: dist5mmM2:4 ↔ AS 1427 H - Metric M2 x 8:20
- Mate:243: RASPBERRY PI 3:1 ↔ AS 1427 H - Metric M2 x 8:17
- Mate:244: RASPBERRY PI 3:1 ↔ AS 1427 H - Metric M2 x 8:18
- Mate:245: RASPBERRY PI 3:1 ↔ AS 1427 H - Metric M2 x 8:19
- Mate:246: RASPBERRY PI 3:1 ↔ AS 1427 H - Metric M2 x 8:20
- Mate:249: top_plate:1 ↔ AS 1112 (2) - Metric M2  Type 5:20
- Mate:250: top_plate:1 ↔ AS 1112 (2) - Metric M2  Type 5:21
- Mate:251: top_plate:1 ↔ AS 1112 (2) - Metric M2  Type 5:22
- Mate:252: top_plate:1 ↔ AS 1112 (2) - Metric M2  Type 5:23
- Mate:253: dist5mmM2:2 ↔ AS 1112 (2) - Metric M2  Type 5:20
- Mate:254: dist5mmM2:5 ↔ AS 1112 (2) - Metric M2  Type 5:21
- Mate:255: dist5mmM2:4 ↔ AS 1112 (2) - Metric M2  Type 5:23
- Mate:256: dist5mmM2:3 ↔ AS 1112 (2) - Metric M2  Type 5:22
- Mate:280: baseplate:1 ↔ dist5mmM2:8
- Mate:281: baseplate:1 ↔ dist5mmM2:7
- Mate:282: baseplate:1 ↔ dist5mmM2:6
- Mate:283: baseplate:1 ↔ dist5mmM2:7
- Mate:284: baseplate:1 ↔ dist5mmM2:6
- Mate:285: baseplate:1 ↔ dist5mmM2:8
- Mate:298: baseplate:1 ↔ AS 1112 (2) - Metric M2  Type 5:24
- Mate:299: baseplate:1 ↔ AS 1112 (2) - Metric M2  Type 5:26
- Mate:300: baseplate:1 ↔ AS 1112 (2) - Metric M2  Type 5:25
- Mate:301: dist5mmM2:7 ↔ AS 1112 (2) - Metric M2  Type 5:26
- Mate:302: dist5mmM2:6 ↔ AS 1112 (2) - Metric M2  Type 5:24
- Mate:303: dist5mmM2:8 ↔ AS 1112 (2) - Metric M2  Type 5:25
- Mate:310: kamera:1 ↔ cam_holder:1
- Mate:311: kamera:1 ↔ cam_holder:1
- Mate:312: kamera:1 ↔ cam_holder:1
- Mate:313: baseplate:1 ↔ cam_holder:1
- Mate:314: baseplate:1 ↔ cam_holder:1
- Mate:315: baseplate:1 ↔ cam_holder:1
- Mate:316: cam_holder:1 ↔ AS 1427 H - Metric M2 x 8:28
- Mate:317: cam_holder:1 ↔ AS 1427 H - Metric M2 x 8:24
- Mate:318: cam_holder:1 ↔ AS 1427 H - Metric M2 x 8:28
- Mate:319: cam_holder:1 ↔ AS 1427 H - Metric M2 x 8:24
- Mate:320: kamera:1 ↔ AS 1427 H - Metric M2 x 8:27
- Mate:321: kamera:1 ↔ AS 1427 H - Metric M2 x 8:27
- Mate:322: kamera:1 ↔ AS 1427 H - Metric M2 x 8:29
- Mate:323: kamera:1 ↔ AS 1427 H - Metric M2 x 8:29
- Mate:324: kamera:1 ↔ AS 1427 H - Metric M2 x 8:26
- Mate:325: kamera:1 ↔ AS 1427 H - Metric M2 x 8:26
- Mate:326: kamera:1 ↔ AS 1427 H - Metric M2 x 8:25
- Mate:327: kamera:1 ↔ AS 1427 H - Metric M2 x 8:25
- Mate:328: baseplate:1 ↔ AS 1112 (2) - Metric M2  Type 5:28
- Mate:329: baseplate:1 ↔ AS 1112 (2) - Metric M2  Type 5:27
- Mate:330: AS 1427 H - Metric M2 x 8:24 ↔ AS 1112 (2) - Metric M2  Type 5:27
- Mate:331: AS 1427 H - Metric M2 x 8:28 ↔ AS 1112 (2) - Metric M2  Type 5:28
- Mate:332: cam_holder:1 ↔ AS 1112 (2) - Metric M2  Type 5:29
- Mate:333: cam_holder:1 ↔ AS 1112 (2) - Metric M2  Type 5:30
- Mate:334: cam_holder:1 ↔ AS 1112 (2) - Metric M2  Type 5:31
- Mate:335: cam_holder:1 ↔ AS 1112 (2) - Metric M2  Type 5:32
- Mate:336: AS 1427 H - Metric M2 x 8:27 ↔ AS 1112 (2) - Metric M2  Type 5:32
- Mate:337: AS 1427 H - Metric M2 x 8:29 ↔ AS 1112 (2) - Metric M2  Type 5:31
- Mate:338: AS 1427 H - Metric M2 x 8:26 ↔ AS 1112 (2) - Metric M2  Type 5:30
- Mate:339: AS 1427 H - Metric M2 x 8:25 ↔ AS 1112 (2) - Metric M2  Type 5:29
- Mate:340: arm_grip:2 ↔ arm_front_rect:1
- Mate:341: arm_grip_mirror:2 ↔ arm_front_rect:2
- Mate:344: arm_grip:1 ↔ arm_back_rect:1
- Mate:345: arm_grip_mirror:1 ↔ arm_back_rect:2
- Mate:346: arm_grip:1 ↔ arm_back_rect:1
- Angle:1 (180 deg): arm_grip:1 ↔ arm_back_rect:1
- Mate:347: arm_grip_mirror:1 ↔ arm_back_rect:2
- Angle:2 (180 deg): arm_grip_mirror:1 ↔ arm_back_rect:2
- Mate:348: arm_grip_mirror:2 ↔ arm_front_rect:2
- Angle:3 (180 deg): arm_grip_mirror:2 ↔ arm_front_rect:2
- Mate:349: arm_grip:2 ↔ arm_front_rect:1
- Angle:4 (180 deg): arm_grip:2 ↔ arm_front_rect:1
- Mate:350: arm_front_rect:1 ↔ motor_mount:1
- Mate:351: arm_front_rect:2 ↔ motor_mount:2
- Mate:352: arm_back_rect:1 ↔ motor_mount:4
- Mate:353: arm_back_rect:2 ↔ motor_mount:3
- Mate:354: arm_back_rect:2 ↔ motor_mount:3
- Mate:355: arm_back_rect:1 ↔ motor_mount:4
- Mate:356: arm_front_rect:1 ↔ motor_mount:1
- Mate:357: arm_front_rect:2 ↔ motor_mount:2
- Angle:5 (0 deg): arm_back_rect:2 ↔ motor_mount:3
- Angle:6 (0 deg): arm_back_rect:1 ↔ motor_mount:4
- Angle:7 (0 deg): arm_front_rect:2 ↔ motor_mount:2
- Angle:8 (0 deg): arm_front_rect:1 ↔ motor_mount:1
- Mate:358: arm_front_rect:2 ↔ motor_mount_lock:1
- Mate:359: motor_mount:2 ↔ motor_mount_lock:1
- Mate:360: motor_mount:2 ↔ motor_mount_lock:1
- Mate:361: arm_front_rect:1 ↔ motor_mount_lock:2
- Mate:362: motor_mount:1 ↔ motor_mount_lock:2
- Mate:363: motor_mount:1 ↔ motor_mount_lock:2
- Mate:364: arm_back_rect:1 ↔ motor_mount_lock:3
- Mate:365: motor_mount:4 ↔ motor_mount_lock:3
- Mate:366: motor_mount:4 ↔ motor_mount_lock:3
- Mate:367: arm_back_rect:2 ↔ motor_mount_lock:4
- Mate:368: motor_mount:3 ↔ motor_mount_lock:4
- Mate:369: motor_mount:3 ↔ motor_mount_lock:4
- Mate:370: motor_mount:1 ↔ Emax Rs2205 v1:2
- Mate:371: arm_front_rect:1 ↔ Emax Rs2205 v1:2
- Mate:372: motor_mount:2 ↔ Emax Rs2205 v1:1
- Mate:373: motor_mount:4 ↔ Emax Rs2205 v1:3
- Mate:374: motor_mount:3 ↔ Emax Rs2205 v1:4
- Mate:375: arm_back_rect:2 ↔ Emax Rs2205 v1:4
- Mate:376: arm_back_rect:1 ↔ Emax Rs2205 v1:3
- Mate:377: arm_front_rect:2 ↔ Emax Rs2205 v1:1
- Mate:378: Emax Rs2205 v1:2 ↔ 5x3_prop:3
- Mate:379: Emax Rs2205 v1:1 ↔ 5x3_prop:2
- Mate:380: Emax Rs2205 v1:4 ↔ 5x3_prop:1
- Mate:381: Emax Rs2205 v1:3 ↔ 5x3_prop:4
- Mate:382 (5 mm): Emax Rs2205 v1:2 ↔ 5x3_prop:3
- Mate:383 (5 mm): Emax Rs2205 v1:3 ↔ 5x3_prop:4
- Mate:384 (5 mm): Emax Rs2205 v1:1 ↔ 5x3_prop:2
- Mate:385 (5 mm): Emax Rs2205 v1:4 ↔ 5x3_prop:1
- Mate:409: baseplate:1 ↔ dist5mmM2:9
- Mate:410: baseplate:1 ↔ dist5mmM2:9
- Mate:412: dist5mmM2:9 ↔ dist10mmM2:12
- Mate:414: dist5mmM2:9 ↔ AS 1427 H - Metric M2 x 8:30
- Mate:415: baseplate:1 ↔ AS 1112 (2) - Metric M2  Type 5:34
- Mate:416: dist5mmM2:9 ↔ AS 1112 (2) - Metric M2  Type 5:34
- Mate:417: baseplate:1 ↔ logic_conventer_lock:1
- Mate:418: baseplate:1 ↔ logic_conventer_lock:1
- Mate:419: top_plate:1 ↔ dist5mmM2:10
- Mate:420: top_plate:1 ↔ dist5mmM2:11
- Mate:421: top_plate:1 ↔ dist5mmM2:10
- Mate:422: top_plate:1 ↔ dist5mmM2:11
- Mate:423: dist5mmM2:11 ↔ AS 1112 (2) - Metric M2  Type 5:35
- Mate:424: dist5mmM2:10 ↔ AS 1112 (2) - Metric M2  Type 5:36
- Mate:425: top_plate:1 ↔ AS 1112 (2) - Metric M2  Type 5:35
- Mate:426: top_plate:1 ↔ AS 1112 (2) - Metric M2  Type 5:36
- Mate:427: altimuv3:1 ↔ dist5mmM2:11
- Mate:428: baseplate:1 ↔ converter:1
- Flush:1: logic_conventer_lock:1 ↔ converter:1
- Mate:429: logic_conventer_lock:1 ↔ converter:1
- Mate:430: baseplate:1 ↔ transformer_mount:1
- Mate:431: baseplate:1 ↔ transformer_mount:1
- Mate:432: baseplate:1 ↔ transformer_mount:2
- Mate:433: baseplate:1 ↔ transformer_mount:2
- Mate:434: transformer_mount:1 ↔ transformer:1
- Mate:435: transformer_mount:1 ↔ transformer:1
- Mate:436: transformer_mount:2 ↔ transformer:1
- Mate:437: baseplate:1 ↔ transformer_mount:3
- Mate:438: baseplate:1 ↔ transformer_mount:4
- Mate:439: baseplate:1 ↔ transformer_mount:3
- Mate:440: baseplate:1 ↔ transformer_mount:4
- Mate:441: transformer_mount:3 ↔ transformer:2
- Mate:442: transformer_mount:3 ↔ transformer:2
- Mate:443: baseplate:1 ↔ dist5mmM2:13
- Mate:444: baseplate:1 ↔ dist5mmM2:15
- Mate:445: baseplate:1 ↔ dist5mmM2:12
- Mate:446: baseplate:1 ↔ dist5mmM2:14
- Mate:447: baseplate:1 ↔ dist5mmM2:13
- Mate:448: baseplate:1 ↔ dist5mmM2:15
- Mate:449: baseplate:1 ↔ dist5mmM2:14
- Mate:450: baseplate:1 ↔ dist5mmM2:12
- Mate:451: baseplate:1 ↔ AS 1112 (2) - Metric M2  Type 5:40
- Mate:452: baseplate:1 ↔ AS 1112 (2) - Metric M2  Type 5:39
- Mate:453: baseplate:1 ↔ AS 1112 (2) - Metric M2  Type 5:38
- Mate:454: baseplate:1 ↔ AS 1112 (2) - Metric M2  Type 5:37
- Mate:455: dist5mmM2:14 ↔ AS 1112 (2) - Metric M2  Type 5:37
- Mate:456: dist5mmM2:13 ↔ AS 1112 (2) - Metric M2  Type 5:40
- Mate:457: dist5mmM2:15 ↔ AS 1112 (2) - Metric M2  Type 5:38
- Mate:458: dist5mmM2:12 ↔ AS 1112 (2) - Metric M2  Type 5:39
- Mate:459: dist5mmM2:6 ↔ regulator:1
- Mate:460: dist10mmM2:12 ↔ regulator:1
- Mate:461: dist10mmM2:9 ↔ regulator:2
- Mate:462: AS 1427 H - Metric M2 x 8:21 ↔ regulator:2
- Mate:463: dist5mmM2:15 ↔ regulator:3
- Mate:464: dist5mmM2:13 ↔ regulator:3
- Mate:465: regulator:3 ↔ dist10mmM2:15
- Mate:466: regulator:3 ↔ dist10mmM2:14
- Mate:467: regulator:3 ↔ dist10mmM2:13
- Mate:468: regulator:3 ↔ dist10mmM2:16
- Mate:469: regulator:3 ↔ dist10mmM2:15
- Mate:470: regulator:3 ↔ dist10mmM2:14
- Mate:471: regulator:3 ↔ dist10mmM2:16
- Mate:472: regulator:3 ↔ dist10mmM2:13
- Mate:473: regulator:4 ↔ dist10mmM2:15
- Mate:474: regulator:4 ↔ dist10mmM2:14
- Mate:475: regulator:4 ↔ dist10mmM2:15
- Mate:476: regulator:4 ↔ AS 1427 H - Metric M2 x 8:32
- Mate:477: regulator:4 ↔ AS 1427 H - Metric M2 x 8:33
- Mate:478: regulator:4 ↔ AS 1427 H - Metric M2 x 8:34
- Mate:479: regulator:4 ↔ AS 1427 H - Metric M2 x 8:31
- Mate:480: regulator:4 ↔ AS 1427 H - Metric M2 x 8:33
- Mate:481: regulator:4 ↔ AS 1427 H - Metric M2 x 8:32
- Mate:482: regulator:4 ↔ AS 1427 H - Metric M2 x 8:34
- Mate:483: regulator:4 ↔ AS 1427 H - Metric M2 x 8:31
- Mate:484: top_plate:1 ↔ dist5mmM2:10
- Mate:485: top_plate:1 ↔ dist5mmM2:11
- Mate:486: altimuv3:1 ↔ dist5mmM2:11
- Mate:487: altimuv3:1 ↔ dist5mmM2:11
- Mate:488: altimuv3:1 ↔ AS 1427 H - Metric M2 x 8:35
- Mate:489: altimuv3:1 ↔ AS 1427 H - Metric M2 x 8:36
- Mate:490: altimuv3:1 ↔ AS 1427 H - Metric M2 x 8:36
- Mate:491: altimuv3:1 ↔ AS 1427 H - Metric M2 x 8:35
- Mate:492: top_plate:1 ↔ AS 1427 H - Metric M2 x 8:39
- Mate:493: top_plate:1 ↔ AS 1427 H - Metric M2 x 8:38
- Mate:494: transformer_mount:3 ↔ AS 1427 H - Metric M2 x 8:40
- Mate:495: transformer_mount:4 ↔ AS 1427 H - Metric M2 x 8:37
- Mate:496: top_plate:1 ↔ AS 1427 H - Metric M2 x 8:43
- Mate:497: top_plate:1 ↔ AS 1427 H - Metric M2 x 8:44
- Mate:498: transformer_mount:2 ↔ AS 1427 H - Metric M2 x 8:42
- Mate:499: transformer_mount:1 ↔ AS 1427 H - Metric M2 x 8:41
- Mate:500: transformer_mount:1 ↔ AS 1427 H - Metric M2 x 8:41
- Mate:501: transformer_mount:2 ↔ AS 1427 H - Metric M2 x 8:42
- Mate:502: top_plate:1 ↔ AS 1427 H - Metric M2 x 8:44
- Mate:503: top_plate:1 ↔ AS 1427 H - Metric M2 x 8:43
- Mate:504: top_plate:1 ↔ AS 1427 H - Metric M2 x 8:39
- Mate:505: top_plate:1 ↔ AS 1427 H - Metric M2 x 8:38
- Mate:506: transformer_mount:3 ↔ AS 1427 H - Metric M2 x 8:40
- Mate:507: transformer_mount:4 ↔ AS 1427 H - Metric M2 x 8:37
- Mate:508: baseplate:1 ↔ AS 1112 (2) - Metric M2  Type 5:41
- Mate:509: baseplate:1 ↔ AS 1112 (2) - Metric M2  Type 5:44
- Mate:510: baseplate:1 ↔ AS 1112 (2) - Metric M2  Type 5:42
- Mate:511: baseplate:1 ↔ AS 1112 (2) - Metric M2  Type 5:43
- Mate:512: AS 1427 H - Metric M2 x 8:41 ↔ AS 1112 (2) - Metric M2  Type 5:43
- Mate:513: AS 1427 H - Metric M2 x 8:42 ↔ AS 1112 (2) - Metric M2  Type 5:44
- Mate:514: AS 1427 H - Metric M2 x 8:37 ↔ AS 1112 (2) - Metric M2  Type 5:41
- Mate:515: AS 1427 H - Metric M2 x 8:40 ↔ AS 1112 (2) - Metric M2  Type 5:42
- Mate:516: transformer_mount:2 ↔ AS 1112 (2) - Metric M2  Type 5:48
- Mate:517: AS 1427 H - Metric M2 x 8:44 ↔ AS 1112 (2) - Metric M2  Type 5:48
- Mate:518: transformer_mount:1 ↔ AS 1112 (2) - Metric M2  Type 5:47
- Mate:519: AS 1427 H - Metric M2 x 8:43 ↔ AS 1112 (2) - Metric M2  Type 5:47
- Mate:520: transformer_mount:3 ↔ AS 1112 (2) - Metric M2  Type 5:46
- Mate:521: AS 1427 H - Metric M2 x 8:39 ↔ AS 1112 (2) - Metric M2  Type 5:46
- Mate:522: transformer_mount:4 ↔ AS 1112 (2) - Metric M2  Type 5:45
- Mate:523: AS 1427 H - Metric M2 x 8:38 ↔ AS 1112 (2) - Metric M2  Type 5:45
- Mate:524: logic_conventer_lock:1 ↔ AS 1427 H - Metric M2 x 8:45
- Mate:525: logic_conventer_lock:1 ↔ AS 1427 H - Metric M2 x 8:46
- Mate:526: logic_conventer_lock:1 ↔ AS 1427 H - Metric M2 x 8:46
- Mate:527: logic_conventer_lock:1 ↔ AS 1427 H - Metric M2 x 8:45
- Mate:528: baseplate:1 ↔ AS 1112 (2) - Metric M2  Type 5:50
- Mate:529: AS 1427 H - Metric M2 x 8:46 ↔ AS 1112 (2) - Metric M2  Type 5:50
- Mate:530: baseplate:1 ↔ AS 1112 (2) - Metric M2  Type 5:49
- Mate:531: AS 1427 H - Metric M2 x 8:45 ↔ AS 1112 (2) - Metric M2  Type 5:49
- Mate:532: baseplate:1 ↔ battery_distancer:1
- Mate:533: baseplate:1 ↔ battery_distancer:1
- Mate:534: baseplate:1 ↔ battery_distancer:1
- Mate:535: baseplate:1 ↔ battery_distancer:2
- Mate:536: baseplate:1 ↔ battery_distancer:2
- Mate:537: baseplate:1 ↔ battery_distancer:2
- Mate:538: baseplate:1 ↔ AS 1427 H - Metric M2 x 8:47
- Mate:539: baseplate:1 ↔ AS 1427 H - Metric M2 x 8:47
- Mate:540: baseplate:1 ↔ AS 1427 H - Metric M2 x 8:48
- Mate:541: baseplate:1 ↔ AS 1427 H - Metric M2 x 8:48
- Mate:542: baseplate:1 ↔ AS 1427 H - Metric M2 x 8:50
- Mate:543: baseplate:1 ↔ AS 1427 H - Metric M2 x 8:49
- Mate:544: baseplate:1 ↔ AS 1427 H - Metric M2 x 8:49
- Mate:545: baseplate:1 ↔ AS 1427 H - Metric M2 x 8:50
- Mate:546: battery_distancer:2 ↔ AS 1112 (2) - Metric M2  Type 5:54
- Mate:547: AS 1427 H - Metric M2 x 8:50 ↔ AS 1112 (2) - Metric M2  Type 5:54
- Mate:548: battery_distancer:1 ↔ AS 1112 (2) - Metric M2  Type 5:53
- Mate:549: AS 1427 H - Metric M2 x 8:49 ↔ AS 1112 (2) - Metric M2  Type 5:53
- Mate:550: battery_distancer:1 ↔ AS 1112 (2) - Metric M2  Type 5:52
- Mate:551: AS 1427 H - Metric M2 x 8:48 ↔ AS 1112 (2) - Metric M2  Type 5:52
- Mate:552: battery_distancer:2 ↔ AS 1112 (2) - Metric M2  Type 5:51
- Mate:553: AS 1427 H - Metric M2 x 8:47 ↔ AS 1112 (2) - Metric M2  Type 5:51
- Mate:554: battery_distancer:2 ↔ battery_vant_4500_4s:1
- Mate:555 (1 mm): battery_distancer:2 ↔ battery_vant_4500_4s:1
- Mate:556: transformer:1 ↔ AS 1427 H - Metric M2 x 8:51
- Mate:557: transformer:1 ↔ AS 1427 H - Metric M2 x 8:52
- Mate:558: transformer:1 ↔ AS 1427 H - Metric M2 x 8:52
- Mate:559: transformer:1 ↔ AS 1427 H - Metric M2 x 8:51
- Mate:560: transformer:2 ↔ AS 1427 H - Metric M2 x 8:54
- Mate:561: transformer:2 ↔ AS 1427 H - Metric M2 x 8:53
- Mate:562: transformer:2 ↔ AS 1427 H - Metric M2 x 8:53
- Mate:563: transformer:2 ↔ AS 1427 H - Metric M2 x 8:54
## Named parameters: sa_0 = -13.8611, sa_1 = 0, sa_2 = 999.904, sa_3 = -5.52663, sa_4 = 0, sa_5 = 999.985, sa_6 = 0, sa_7 = -500, sa_8 = -0
note: some values were not read from the file. Shown as the stored number, unit unknown: "sa_0", "sa_1", "sa_2", "sa_3", "sa_4", "sa_5", "sa_6", "sa_7", "sa_8".
